# Autodesk Inventor assembly: connecting_rod_sub_Assembly
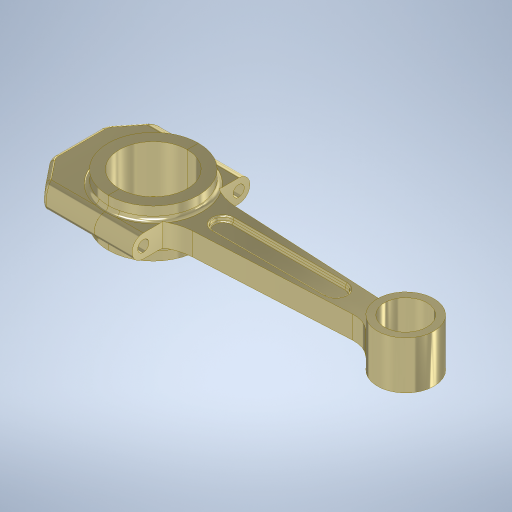
[picture p0: Inventor's stored thumbnail of the model, 512x512]
Saved by Autodesk Inventor 2023 (Build 270158000, 158)
## iProperties
Created: 2023-10-21
Part Number: connecting_rod_sub_Assembly
Document SubType Name: Assembly
Designer: Beatrice
Author: Beatrice
## Documents named in this file (3)
- C:\Users\Beatrice\Documents\Inventor\4_Cylinder_Engine\4 cylinder engine assembly\connecting_rod_sub_Assembly.iam
- C:\Users\Beatrice\Documents\Inventor\4_Cylinder_Engine\4 cylinder engine assembly\connecting rod.ipt
- C:\Users\Beatrice\Documents\Inventor\4_Cylinder_Engine\4 cylinder engine assembly\connecting rod_cap.ipt
## Components (2 placed, 2 different names)
1. connecting rod:1 — Insert:1, Insert:2
2. connecting rod_cap:1 — Insert:1, Insert:2
## Relationships (2: Insert 2)
- Insert:1: connecting rod:1 ↔ connecting rod_cap:1
- Insert:2: connecting rod:1 ↔ connecting rod_cap:1
